# Autodesk Inventor assembly: base
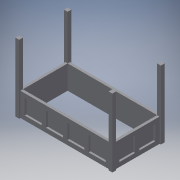
[picture p0: Inventor's stored thumbnail of the model, 180x180]
Saved by Autodesk Inventor 2017 (Build 210142000, 142)
## iProperties
Created: 2019-05-05
Part Number: base
Document SubType Name: Assembly
Designer: Roman
Author: Roman
## Documents named in this file (4)
- C:\Users\Roman\Documents\CAD\tegu rev2\base\base.iam
- C:\Users\Roman\Documents\CAD\tegu rev2\base\short wall\base short wall.iam
- C:\Users\Roman\Documents\CAD\tegu rev2\base\long wall\base long wall.iam
- C:\Users\Roman\Documents\CAD\tegu rev2\base\base pillar.ipt
## Components (8 placed, 3 different names)
1. base short wall:1 [sub-assembly] — Mate:4, Flush:8, Mate:5, Flush:10, Flush:17, Flush:21
2. base short wall:2 [sub-assembly] — Mate:3, Flush:6, Mate:6, Flush:12, Flush:18, Flush:19
3. base long wall:1 [sub-assembly] — Flush:1, Mate:1, Mate:2, Flush:4, Flush:15, Flush:16
4. base long wall:2 [sub-assembly] — Flush:14, Mate:7, Flush:20
5. base pillar:1 — Mate:6, Flush:12, Flush:14, Mate:7, Flush:19, Flush:20
6. base pillar:2 — Mate:5, Flush:10, Flush:21
7. base pillar:3 — Flush:1, Mate:1, Mate:4, Flush:8, Flush:16, Flush:17
8. base pillar:4 — Mate:2, Flush:4, Mate:3, Flush:6, Flush:15, Flush:18
## Relationships (21: Flush 14, Mate 7)
- Flush:1: base long wall:1 ↔ base pillar:3
- Mate:1: base long wall:1 ↔ base pillar:3
- Mate:2: base long wall:1 ↔ base pillar:4
- Flush:4: base long wall:1 ↔ base pillar:4
- Mate:3: base short wall:2 ↔ base pillar:4
- Flush:6: base short wall:2 ↔ base pillar:4
- Mate:4: base short wall:1 ↔ base pillar:3
- Flush:8: base short wall:1 ↔ base pillar:3
- Mate:5: base short wall:1 ↔ base pillar:2
- Flush:10: base short wall:1 ↔ base pillar:2
- Mate:6: base short wall:2 ↔ base pillar:1
- Flush:12: base short wall:2 ↔ base pillar:1
- Flush:14: base long wall:2 ↔ base pillar:1
- Mate:7: base long wall:2 ↔ base pillar:1
- Flush:15: base long wall:1 ↔ base pillar:4
- Flush:16: base long wall:1 ↔ base pillar:3
- Flush:17: base short wall:1 ↔ base pillar:3
- Flush:18: base short wall:2 ↔ base pillar:4
- Flush:19: base short wall:2 ↔ base pillar:1
- Flush:20: base long wall:2 ↔ base pillar:1
- Flush:21: base short wall:1 ↔ base pillar:2
